# Autodesk Inventor assembly: RC5
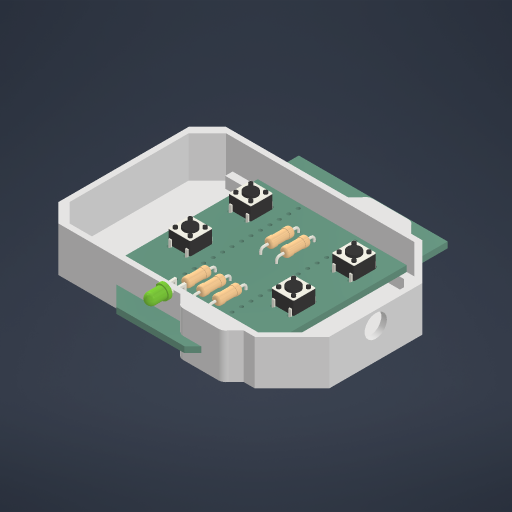
[picture p0: Inventor's stored thumbnail of the model, 512x512]
Saved by Autodesk Inventor 2024 (Build 280153000, 153)
## iProperties
Created: 2024-03-14
Part Number: RC5
Document SubType Name: Assembly
Designer: MenMe
Author: MenMe
## Documents named in this file (4)
- C:\Users\Simak\OneDrive\Dokumenty\GitHub\RoboCop\- 3D -\other\RC5.iam
- C:\Users\Simak\OneDrive\Dokumenty\GitHub\RoboCop\- 3D -\other\RC5 Controller.ipt
- C:\Users\Simak\OneDrive\Dokumenty\GitHub\RoboCop\- 3D -\other\RC5 Controller kryt.ipt
- C:\Users\Simak\OneDrive\Dokumenty\GitHub\RoboCop\- 3D -\PCBs\RC5 Remote\RC-5 Remote Controler\RC-5 Remote Controler.iam
## Components (3 placed, 3 different names)
1. RC5 Controller:1 — Proti sobě:3, Proti sobě:4, Proti sobě:5, Proti sobě:6
2. RC5 Controller kryt:1 — Proti sobě:3, Proti sobě:4, Proti sobě:5
3. RC-5 Remote Controler:1 [sub-assembly] — Proti sobě:6
## Relationships (4: Mate 4)
- Proti sobě:3 [Mate]: RC5 Controller:1 ↔ RC5 Controller kryt:1
- Proti sobě:4 [Mate]: RC5 Controller:1 ↔ RC5 Controller kryt:1
- Proti sobě:5 [Mate]: RC5 Controller:1 ↔ RC5 Controller kryt:1
- Proti sobě:6 [Mate]: RC5 Controller:1 ↔ RC-5 Remote Controler:1
